# Autodesk Inventor assembly: base-weel-2
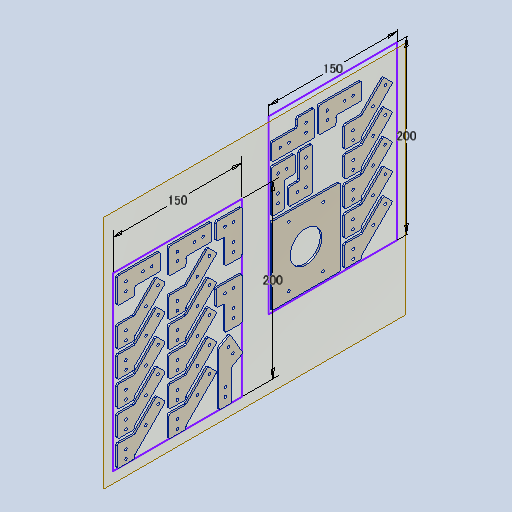
[picture p0: Inventor's stored thumbnail of the model, 512x512]
Saved by Autodesk Inventor 2025.2 (Build 292293000, 293)
## iProperties
Created: 2025-01-14
Part Number: base-weel-2
Document SubType Name: Assembly
Designer: haruy
Author: haruy
## Documents named in this file (6)
- C:\Users\haruy\Documents\ロボコン\NHK2025\cad\cnc\base-weel-2.iam
- C:\Users\haruy\Documents\ロボコン\NHK2025\cad\nagahisa\base_weel\base_weel-v2-Plate-3.ipt
- C:\Users\haruy\Documents\ロボコン\NHK2025\cad\nagahisa\base_weel\base_weel-v2-Plate-4.ipt
- C:\Users\haruy\Documents\ロボコン\NHK2025\cad\nagahisa\base_weel\base_weel-v2-Plate-1.ipt
- C:\Users\haruy\Documents\ロボコン\NHK2025\cad\nagahisa\base_weel\base_weel-v2-Plate-8.ipt
- C:\Users\haruy\Documents\ロボコン\NHK2025\cad\nagahisa\belt_liner\belt_liner_v2_Plate_20.ipt
## Components (25 placed, 5 different names)
1. base_weel-v2-Plate-1:1 — フラッシュ:9, フラッシュ:21, メイト:2, メイト:3, フラッシュ:24
2. base_weel-v2-Plate-8:1 — フラッシュ:22, フラッシュ:23, メイト:4
3. base_weel-v2-Plate-8:4 — フラッシュ:13, フラッシュ:23, メイト:3, フラッシュ:24, メイト:4, フラッシュ:28, メイト:5
4. belt_liner_v2_Plate_20:2 — フラッシュ:15, フラッシュ:17
5. base_weel-v2-Plate-4:3 — フラッシュ:18, 角度:1, フラッシュ:19, フラッシュ:20
6. base_weel-v2-Plate-4:4 — フラッシュ:19, フラッシュ:20
7. base_weel-v2-Plate-4:5 — フラッシュ:25, メイト:6, フラッシュ:29
8. base_weel-v2-Plate-4:6 — フラッシュ:27, フラッシュ:28, メイト:5, メイト:6, フラッシュ:29
9. base_weel-v2-Plate-3:1 — フラッシュ:1, フラッシュ:3, メイト:1
10. base_weel-v2-Plate-3:7 — フラッシュ:17
11. base_weel-v2-Plate-4:1 — フラッシュ:7, フラッシュ:8
12. base_weel-v2-Plate-4:2 — 角度:1
13. base_weel-v2-Plate-3:17 — フラッシュ:4, フラッシュ:21, メイト:2
14. base_weel-v2-Plate-3:18
15. base_weel-v2-Plate-3:19
16. base_weel-v2-Plate-3:20
17. base_weel-v2-Plate-3:21
18. base_weel-v2-Plate-3:2 — フラッシュ:2, フラッシュ:3, メイト:1
19. base_weel-v2-Plate-3:4
20. base_weel-v2-Plate-3:5
21. base_weel-v2-Plate-3:6 — フラッシュ:8
22. base_weel-v2-Plate-3:8
23. base_weel-v2-Plate-3:9
24. base_weel-v2-Plate-3:10
25. base_weel-v2-Plate-3:11
## Component patterns: (3 elements, first: base_weel-v2-Plate-3:1), (4 elements, first: base_weel-v2-Plate-4:1), (5 elements, first: base_weel-v2-Plate-3:17), (4 elements, first: base_weel-v2-Plate-3:2), コンポーネント パターン 1:2 (4 elements)
## Relationships (28: Flush 21, Mate 6, Angle 1)
- フラッシュ:1 [Flush]: base_weel-v2-Plate-3:1
- フラッシュ:2 [Flush]: base_weel-v2-Plate-3:2
- フラッシュ:3 [Flush]: base_weel-v2-Plate-3:1 ↔ base_weel-v2-Plate-3:2
- メイト:1 [Mate] (5 mm): base_weel-v2-Plate-3:1 ↔ base_weel-v2-Plate-3:2
- フラッシュ:4 [Flush]: base_weel-v2-Plate-3:17
- フラッシュ:7 [Flush]: base_weel-v2-Plate-4:1
- フラッシュ:8 [Flush]: base_weel-v2-Plate-4:1 ↔ base_weel-v2-Plate-3:6
- フラッシュ:9 [Flush]: base_weel-v2-Plate-1:1
- フラッシュ:13 [Flush]: base_weel-v2-Plate-8:4
- フラッシュ:15 [Flush]: belt_liner_v2_Plate_20:2
- フラッシュ:17 [Flush]: belt_liner_v2_Plate_20:2 ↔ base_weel-v2-Plate-3:7
- フラッシュ:18 [Flush]: base_weel-v2-Plate-4:3
- 角度:1 [Angle] (0 deg): base_weel-v2-Plate-4:3 ↔ base_weel-v2-Plate-4:2
- フラッシュ:19 [Flush]: base_weel-v2-Plate-4:3 ↔ base_weel-v2-Plate-4:4
- フラッシュ:20 [Flush]: base_weel-v2-Plate-4:3 ↔ base_weel-v2-Plate-4:4
- フラッシュ:21 [Flush]: base_weel-v2-Plate-1:1 ↔ base_weel-v2-Plate-3:17
- メイト:2 [Mate] (5 mm): base_weel-v2-Plate-1:1 ↔ base_weel-v2-Plate-3:17
- フラッシュ:22 [Flush]: base_weel-v2-Plate-8:1
- フラッシュ:23 [Flush]: base_weel-v2-Plate-8:1 ↔ base_weel-v2-Plate-8:4
- メイト:3 [Mate] (5 mm): base_weel-v2-Plate-1:1 ↔ base_weel-v2-Plate-8:4
- フラッシュ:24 [Flush]: base_weel-v2-Plate-1:1 ↔ base_weel-v2-Plate-8:4
- メイト:4 [Mate] (5 mm): base_weel-v2-Plate-8:1 ↔ base_weel-v2-Plate-8:4
- フラッシュ:25 [Flush]: base_weel-v2-Plate-4:5
- フラッシュ:27 [Flush]: base_weel-v2-Plate-4:6
- フラッシュ:28 [Flush]: base_weel-v2-Plate-8:4 ↔ base_weel-v2-Plate-4:6
- メイト:5 [Mate] (5 mm): base_weel-v2-Plate-8:4 ↔ base_weel-v2-Plate-4:6
- メイト:6 [Mate] (5 mm): base_weel-v2-Plate-4:5 ↔ base_weel-v2-Plate-4:6
- フラッシュ:29 [Flush]: base_weel-v2-Plate-4:5 ↔ base_weel-v2-Plate-4:6
